# Autodesk Inventor assembly: VANT_ASSEMBLY
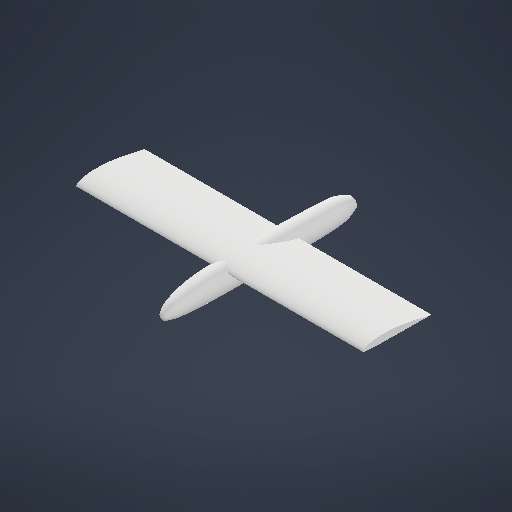
[picture p0: Inventor's stored thumbnail of the model, 512x512]
Saved by Autodesk Inventor 2026.1 (Build 301233000, 233)
## iProperties
Created: 2026-06-28
Part Number: VANT_ASSEMBLY
Document SubType Name: Assembly
Designer: adria
Author: adria
## Documents named in this file (3)
- C:\Users\adria\Desktop\VANT\VANT_ASSEMBLY.iam
- C:\Users\adria\Desktop\VANT\Airfoil.ipt
- C:\Users\adria\Desktop\VANT\Main_Body.ipt
## Components (2 placed, 2 different names)
1. Airfoil:1 — Flush:1, Mate:1, Angle:1
2. Main_Body:1 — Flush:2, Flush:3, Flush:4, Mate:1
## Relationships (6: Flush 4, Mate 1, Angle 1)
- Flush:1: Airfoil:1
- Flush:2: Main_Body:1
- Flush:3: Main_Body:1
- Flush:4: Main_Body:1
- Mate:1 (-330 mm): Airfoil:1 ↔ Main_Body:1
- Angle:1 (2 deg): Airfoil:1
